# Autodesk Inventor assembly: ToASI-0A
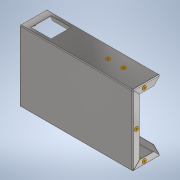
[picture p0: Inventor's stored thumbnail of the model, 180x180]
Saved by Autodesk Inventor 2020.3 (Build 243373000, 373)
## iProperties
Created: 2020-07-31
Part Number: ToASI-0A
Document SubType Name: Assembly
Designer: Bruno
Author: Bruno
## Documents named in this file (3)
- C:\Users\Bruno\Desktop\Github\CAD\Inventor\For ASI\ToASI-0A.iam
- C:\Users\Bruno\Desktop\Github\CAD\Inventor\Heater-Box\Box-Disk\Box base.ipt
- C:\Users\Bruno\Desktop\Github\CAD\Inventor\Heater-Box\Box-Disk\M4 Rivet nut.ipt
## Components (13 placed, 2 different names)
1. Box base:1 — Cylindrical:1, Cylindrical:2, Cylindrical:3, Cylindrical:4, Cylindrical:5, Cylindrical:6, Cylindrical:7, Cylindrical:8, Cylindrical:9, Rotational:1, Rotational:2, Rotational:3
2. M4 Rivet nut:1 — Cylindrical:6
3. M4 Rivet nut:2 — Cylindrical:7
4. M4 Rivet nut:3 — Cylindrical:8
5. M4 Rivet nut:4 — Cylindrical:9
6. M4 Rivet nut:5 — Cylindrical:4
7. M4 Rivet nut:6 — Cylindrical:5
8. M4 Rivet nut:7 — Cylindrical:3
9. M4 Rivet nut:8 — Rotational:3
10. M4 Rivet nut:9 — Rotational:2
11. M4 Rivet nut:10 — Rotational:1
12. M4 Rivet nut:11 — Cylindrical:1
13. M4 Rivet nut:12 — Cylindrical:2
## Relationships (12: CylindricalJoint 9, RevoluteJoint 3)
- Cylindrical:1: Box base:1 ↔ M4 Rivet nut:11
- Cylindrical:2: Box base:1 ↔ M4 Rivet nut:12
- Cylindrical:3: Box base:1 ↔ M4 Rivet nut:7
- Cylindrical:4: Box base:1 ↔ M4 Rivet nut:5
- Cylindrical:5: Box base:1 ↔ M4 Rivet nut:6
- Cylindrical:6: Box base:1 ↔ M4 Rivet nut:1
- Cylindrical:7: Box base:1 ↔ M4 Rivet nut:2
- Cylindrical:8: Box base:1 ↔ M4 Rivet nut:3
- Cylindrical:9: Box base:1 ↔ M4 Rivet nut:4
- Rotational:1 [RevoluteJoint]: Box base:1 ↔ M4 Rivet nut:10
- Rotational:2 [RevoluteJoint]: Box base:1 ↔ M4 Rivet nut:9
- Rotational:3 [RevoluteJoint]: Box base:1 ↔ M4 Rivet nut:8
